# Autodesk Inventor assembly: threadTest
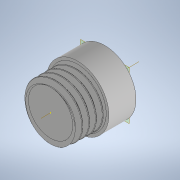
[picture p0: Inventor's stored thumbnail of the model, 180x180]
Saved by Autodesk Inventor 2022 (Build 260153000, 153)
## iProperties
Created: 2021-10-07
Part Number: threadTest
Document SubType Name: Assembly
Designer: tecware
Author: tecware
## Documents named in this file (3)
- C:\Users\tecware\Documents\Inventor\activeMarker\wand\T Clamp and Pipe Extension\threadTest.iam
- C:\Users\tecware\Documents\Inventor\activeMarker\wand\T Clamp and Pipe Extension\threadTeset.ipt
- C:\Users\tecware\Documents\Inventor\activeMarker\wand\T Clamp and Pipe Extension\threadTest-f.ipt
## Components (2 placed, 2 different names)
1. threadTeset:1 — Flush:1
2. threadTest-f:1 — Flush:1
## Relationships (1: Flush 1)
- Flush:1: threadTeset:1 ↔ threadTest-f:1
